# Autodesk Inventor assembly: X-axis Y-axis Motor Holder assy
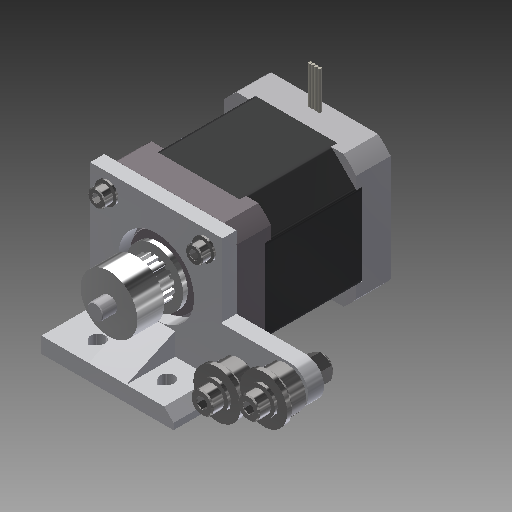
[picture p0: Inventor's stored thumbnail of the model, 512x512]
Saved by Autodesk Inventor 2018 (Build 220112000, 112)
## iProperties
Created: 2017-10-03
Part Number: X-axis Y-axis Motor Holder assy
Document SubType Name: Assembly
Designer: Gabriel Smolnycki
Author: Gabriel Smolnycki
## Documents named in this file (11)
- E:\planb\mechanics\V1INV\Subassemblies\X-axis Y-axis Motor Holder assy.iam
- E:\planb\mechanics\V1INV\X-axis\X-axis Y Motor Holder.ipt
- E:\planb\mechanics\V1INV\Electronics\ST4118L1804-A.ipt
- E:\planb\mechanics\V1INV\Hardware\M3 SS Washer.ipt
- E:\planb\mechanics\V1INV\Hardware\M3x10 SS SHCS.ipt
- E:\planb\mechanics\V1INV\Hardware\T2.5 16T Pulley.ipt
- E:\planb\mechanics\V1INV\Hardware\M4 SS Washer.ipt
- E:\planb\mechanics\V1INV\Hardware\M4 SS Locknut.ipt
- E:\planb\mechanics\V1INV\Hardware\4x13 SS Ball Bearing (7804K103).ipt
- E:\planb\mechanics\V1INV\Hardware\M5 SS Fender Washer.ipt
- E:\planb\mechanics\V1INV\Hardware\M4x20 SS SHCS.ipt
## Components (25 placed, 10 different names)
1. X-axis Y Motor Holder:1 — Insert:1, Insert:2, Insert:3, Insert:4, Insert:5, Insert:10, Insert:11, Insert:12, Insert:13
2. ST4118L1804-A:1 — Insert:1, Insert:2, Insert:9
3. M3 SS Washer:1 — Insert:3, Insert:7
4. M3 SS Washer:2 — Insert:4, Insert:6
5. M3 SS Washer:3 — Insert:5, Insert:8
6. M3x10 SS SHCS:1 — Insert:6
7. M3x10 SS SHCS:2 — Insert:7
8. M3x10 SS SHCS:3 — Insert:8
9. T2.5 16T Pulley:1 — Insert:9
10. M4 SS Washer:1 — Insert:13, Insert:15
11. M4 SS Washer:2 — Insert:12, Insert:14
12. M4 SS Washer:3 — Insert:11, Insert:17
13. M4 SS Washer:4 — Insert:10, Insert:16
14. M4 SS Washer:5 — Insert:19, Insert:21
15. M4 SS Washer:6 — Insert:18, Insert:20
16. M4 SS Washer:7 — Insert:23, Insert:25
17. M4 SS Washer:8 — Insert:22, Insert:24
18. M4 SS Locknut:1 — Insert:14
19. M4 SS Locknut:2 — Insert:15
20. 4x13 SS Ball Bearing (7804K103):1 — Insert:16, Insert:18
21. 4x13 SS Ball Bearing (7804K103):2 — Insert:17, Insert:19
22. M5 SS Fender Washer:1 — Insert:20, Insert:22
23. M5 SS Fender Washer:2 — Insert:21, Insert:23
24. M4x20 SS SHCS:1 — Insert:25
25. M4x20 SS SHCS:2 — Insert:24
## Relationships (25: Insert 25)
- Insert:1: X-axis Y Motor Holder:1 ↔ ST4118L1804-A:1
- Insert:2: X-axis Y Motor Holder:1 ↔ ST4118L1804-A:1
- Insert:3: X-axis Y Motor Holder:1 ↔ M3 SS Washer:1
- Insert:4: X-axis Y Motor Holder:1 ↔ M3 SS Washer:2
- Insert:5: X-axis Y Motor Holder:1 ↔ M3 SS Washer:3
- Insert:6: M3 SS Washer:2 ↔ M3x10 SS SHCS:1
- Insert:7: M3 SS Washer:1 ↔ M3x10 SS SHCS:2
- Insert:8: M3 SS Washer:3 ↔ M3x10 SS SHCS:3
- Insert:9 (4.5 mm): ST4118L1804-A:1 ↔ T2.5 16T Pulley:1
- Insert:10: X-axis Y Motor Holder:1 ↔ M4 SS Washer:4
- Insert:11: X-axis Y Motor Holder:1 ↔ M4 SS Washer:3
- Insert:12: X-axis Y Motor Holder:1 ↔ M4 SS Washer:2
- Insert:13: X-axis Y Motor Holder:1 ↔ M4 SS Washer:1
- Insert:14: M4 SS Washer:2 ↔ M4 SS Locknut:1
- Insert:15: M4 SS Washer:1 ↔ M4 SS Locknut:2
- Insert:16: M4 SS Washer:4 ↔ 4x13 SS Ball Bearing (7804K103):1
- Insert:17: M4 SS Washer:3 ↔ 4x13 SS Ball Bearing (7804K103):2
- Insert:18: M4 SS Washer:6 ↔ 4x13 SS Ball Bearing (7804K103):1
- Insert:19: M4 SS Washer:5 ↔ 4x13 SS Ball Bearing (7804K103):2
- Insert:20: M4 SS Washer:6 ↔ M5 SS Fender Washer:1
- Insert:21: M4 SS Washer:5 ↔ M5 SS Fender Washer:2
- Insert:22: M4 SS Washer:8 ↔ M5 SS Fender Washer:1
- Insert:23: M4 SS Washer:7 ↔ M5 SS Fender Washer:2
- Insert:24: M4 SS Washer:8 ↔ M4x20 SS SHCS:2
- Insert:25: M4 SS Washer:7 ↔ M4x20 SS SHCS:1
